# Autodesk Inventor assembly: Шафа силовая
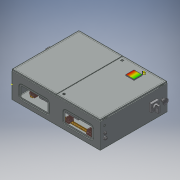
[picture p0: Inventor's stored thumbnail of the model, 180x180]
Saved by Autodesk Inventor 2018 (Build 220112000, 112)
## iProperties
Created: 2018-12-14
Part Number: Шафа силовая
Material: Типовые
Document SubType Name: Assembly
Designer: A.Vlaschuk
Author: A.Vlaschuk
## Documents named in this file (13)
- D:\Проекти\01 Модернизация стенда гидроамортизаторов\КД\STAS60\Шафа силовая.iam
- D:\Проекти\01 Модернизация стенда гидроамортизаторов\КД\STAS60\RITTAL_USA_AE11305002\AIS2018\1130_01_00 (2).ipt
- D:\Проекти\01 Модернизация стенда гидроамортизаторов\КД\STAS60\RITTAL_USA_AE11305002\AIS2018\1130_01_03 (2).ipt
- D:\Проекти\01 Модернизация стенда гидроамортизаторов\КД\STAS60\RITTAL_USA_AE11305002\AIS2018\1XXX_01_04.ipt
- D:\Проекти\01 Модернизация стенда гидроамортизаторов\КД\STAS60\PG13.5\SKINTOP ST PG 13,5      Art_ Nr_ 53015030(F=5)_Kunststoff.ipt
- D:\Проекти\01 Модернизация стенда гидроамортизаторов\КД\STAS60\PG16.0\SKINTOP ST PG 16      Art_ Nr_ 53015240(F=9)_Kunststoff.ipt
- D:\Проекти\01 Модернизация стенда гидроамортизаторов\КД\STAS60\Монтажная панель 19_11_2018.iam
- D:\Проекти\01 Модернизация стенда гидроамортизаторов\КД\STAS60\CAD Eaton\NZM1-XS-R\AIS2018\100031(5,310)_P1.ipt
- D:\Проекти\01 Модернизация стенда гидроамортизаторов\КД\STAS60\PG21\SKINTOP ST PG 21      Art_ Nr_ 53015050(F=13)_Kunststoff.ipt
- D:\Проекти\01 Модернизация стенда гидроамортизаторов\КД\STAS60\CAD Eaton\M22-PVL60P (152861)\152861.ipt
- D:\Проекти\01 Модернизация стенда гидроамортизаторов\КД\STAS60\din-Rail socket\2963491.ipt
- D:\Проекти\01 Модернизация стенда гидроамортизаторов\КД\STAS60\CAD Eaton\EM20.ipt
- D:\Проекти\01 Модернизация стенда гидроамортизаторов\КД\STAS60\RITTAL_USA_AE11305002\AIS2018\1130_01_02 (2).ipt
## Components (22 placed, 12 different names)
1. 1130_01_00 (2):1 — Совмещение:1, Совмещение:2, Совмещение:3, Совмещение:4, Заподлицо:1, Заподлицо:3, Заподлицо:5, Заподлицо:6, Совмещение:5, Вставка:6, Совмещение:6, Совмещение:7, Совмещение:8, Совмещение:9, Совмещение:10, Совмещение:11, Совмещение:12, Совмещение:13, Совмещение:14, Совмещение:15, Заподлицо:7
2. 1XXX_01_04:1 — Совмещение:1, Заподлицо:1, Вставка:3, Заподлицо:5
3. 1XXX_01_04:2 — Совмещение:2, Вставка:2
4. 1XXX_01_04:3 — Совмещение:3, Заподлицо:3
5. 1XXX_01_04:4 — Совмещение:4, Заподлицо:6, Заподлицо:7, Вставка:7
6. 1130_01_03 (2):1 — Вставка:2, Вставка:3, Совмещение:16, Совмещение:17, Совмещение:18
7. SKINTOP ST PG 16      Art_ Nr_ 53015240(F=9)_Kunststoff:1 — Совмещение:6, Совмещение:7
8. Монтажная панель 19_11_2018:1 [sub-assembly] — Совмещение:8
9. 100031(5,310)_P1:1 — Совмещение:9, Совмещение:10
10. SKINTOP ST PG 21      Art_ Nr_ 53015050(F=13)_Kunststoff:1 — Совмещение:11, Совмещение:12
11. 152861:1 — Совмещение:13, Совмещение:14
12. 2963491:1 — Совмещение:15
13. EM20:1 — Совмещение:16, Совмещение:17, Совмещение:18
14. 1130_01_02 (2):1 — Вставка:7
15. SKINTOP ST PG 13,5      Art_ Nr_ 53015030(F=5)_Kunststoff:1 — Совмещение:5, Вставка:6
16. SKINTOP ST PG 13,5      Art_ Nr_ 53015030(F=5)_Kunststoff:2
17. SKINTOP ST PG 13,5      Art_ Nr_ 53015030(F=5)_Kunststoff:3
18. SKINTOP ST PG 13,5      Art_ Nr_ 53015030(F=5)_Kunststoff:4
19. SKINTOP ST PG 13,5      Art_ Nr_ 53015030(F=5)_Kunststoff:5
20. SKINTOP ST PG 13,5      Art_ Nr_ 53015030(F=5)_Kunststoff:6
21. SKINTOP ST PG 13,5      Art_ Nr_ 53015030(F=5)_Kunststoff:7
22. SKINTOP ST PG 13,5      Art_ Nr_ 53015030(F=5)_Kunststoff:8
## Component patterns: (8 elements, first: SKINTOP ST PG 13,5      Art_ Nr_ 53015030(F=5)_Kunststoff:1)
## Relationships (27: Mate 18, Flush 5, Insert 4)
- Совмещение:1 [Mate]: 1130_01_00 (2):1 ↔ 1XXX_01_04:1
- Совмещение:2 [Mate]: 1130_01_00 (2):1 ↔ 1XXX_01_04:2
- Совмещение:3 [Mate]: 1130_01_00 (2):1 ↔ 1XXX_01_04:3
- Совмещение:4 [Mate]: 1130_01_00 (2):1 ↔ 1XXX_01_04:4
- Заподлицо:1 [Flush] (5 mm): 1130_01_00 (2):1 ↔ 1XXX_01_04:1
- Заподлицо:3 [Flush] (5 mm): 1130_01_00 (2):1 ↔ 1XXX_01_04:3
- Вставка:2 [Insert]: 1XXX_01_04:2 ↔ 1130_01_03 (2):1
- Вставка:3 [Insert]: 1XXX_01_04:1 ↔ 1130_01_03 (2):1
- Заподлицо:5 [Flush] (30 mm): 1130_01_00 (2):1 ↔ 1XXX_01_04:1
- Заподлицо:6 [Flush] (30 mm): 1130_01_00 (2):1 ↔ 1XXX_01_04:4
- Совмещение:5 [Mate]: 1130_01_00 (2):1 ↔ SKINTOP ST PG 13,5      Art_ Nr_ 53015030(F=5)_Kunststoff:1
- Вставка:6 [Insert]: 1130_01_00 (2):1 ↔ SKINTOP ST PG 13,5      Art_ Nr_ 53015030(F=5)_Kunststoff:1
- Совмещение:6 [Mate]: 1130_01_00 (2):1 ↔ SKINTOP ST PG 16      Art_ Nr_ 53015240(F=9)_Kunststoff:1
- Совмещение:7 [Mate]: 1130_01_00 (2):1 ↔ SKINTOP ST PG 16      Art_ Nr_ 53015240(F=9)_Kunststoff:1
- Совмещение:8 [Mate] (10 mm): 1130_01_00 (2):1 ↔ Монтажная панель 19_11_2018:1
- Совмещение:9 [Mate]: 1130_01_00 (2):1 ↔ 100031(5,310)_P1:1
- Совмещение:10 [Mate]: 1130_01_00 (2):1 ↔ 100031(5,310)_P1:1
- Совмещение:11 [Mate]: 1130_01_00 (2):1 ↔ SKINTOP ST PG 21      Art_ Nr_ 53015050(F=13)_Kunststoff:1
- Совмещение:12 [Mate]: 1130_01_00 (2):1 ↔ SKINTOP ST PG 21      Art_ Nr_ 53015050(F=13)_Kunststoff:1
- Совмещение:13 [Mate]: 1130_01_00 (2):1 ↔ 152861:1
- Совмещение:14 [Mate]: 1130_01_00 (2):1 ↔ 152861:1
- Совмещение:15 [Mate]: 1130_01_00 (2):1 ↔ 2963491:1
- Совмещение:16 [Mate]: 1130_01_03 (2):1 ↔ EM20:1
- Совмещение:17 [Mate]: 1130_01_03 (2):1 ↔ EM20:1
- Совмещение:18 [Mate]: 1130_01_03 (2):1 ↔ EM20:1
- Заподлицо:7 [Flush] (5 mm): 1130_01_00 (2):1 ↔ 1XXX_01_04:4
- Вставка:7 [Insert]: 1XXX_01_04:4 ↔ 1130_01_02 (2):1
